# Autodesk Inventor assembly: 00_025_SHOE_R1
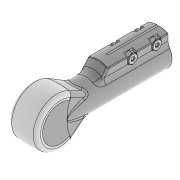
[picture p0: Inventor's stored thumbnail of the model, 180x180]
Saved by Autodesk Inventor 2021.2 (Build 252289000, 289)
## iProperties
Created: 2020-02-11
Part Number: 00_025_SHOE_R1
Material: 一般
Document SubType Name: Assembly
Designer: y6tada
Mass: 6.94447 g
Surface Area: 43.5356 cm^2
Volume: 6.21509 cm^3
Density: 1.11736 g/cm^3
Author: y6tada
## Documents named in this file (5)
- C:\Workspace\HaptHexa\Hardware\Inventor\00_025_SHOE_R1.iam
- C:\Workspace\HaptHexa\Hardware\Inventor\15_026_SHOE_GRIP_BASE_R3.ipt
- C:\Workspace\HaptHexa\Hardware\Inventor\11_027_SHOE_GRIP_RUBBER_R1.ipt
- C:\Users\y6tada\Documents\Inventor\Content Center Files\R2021\en-US\JIS B 1176\JIS B 1176 - M2 x 8 - 0.4.ipt
- C:\Workspace\HaptHexa\Hardware\Inventor\10_028_NYLON_NUT_M2_R1.ipt
## Components (6 placed, 4 different names)
1. GRIP_BASE_V2:1 — Insert:1, Insert:2, Insert:3, Insert:4, Angle:1, Angle:2
2. GRIP_RUBBER:1 — フラッシュ:1
3. JIS B 1176 - Metric M2 x 8:1 — Insert:1
4. JIS B 1176 - Metric M2 x 8:2 — Insert:2
5. NYLOC_NUT_M2:1 — Insert:3, Angle:1
6. NYLOC_NUT_M2:2 — Insert:4, Angle:2
## Relationships (7: Insert 4, Angle 2, Flush 1)
- フラッシュ:1 [Flush]: GRIP_RUBBER:1
- Insert:1: GRIP_BASE_V2:1 ↔ JIS B 1176 - Metric M2 x 8:1
- Insert:2: GRIP_BASE_V2:1 ↔ JIS B 1176 - Metric M2 x 8:2
- Insert:3: GRIP_BASE_V2:1 ↔ NYLOC_NUT_M2:1
- Insert:4: GRIP_BASE_V2:1 ↔ NYLOC_NUT_M2:2
- Angle:1 (0 deg): GRIP_BASE_V2:1 ↔ NYLOC_NUT_M2:1
- Angle:2 (0 deg): GRIP_BASE_V2:1 ↔ NYLOC_NUT_M2:2
